# Autodesk Inventor assembly: Пустой корпус
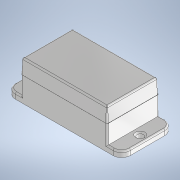
[picture p0: Inventor's stored thumbnail of the model, 180x180]
Saved by Autodesk Inventor 2022 (Build 260153000, 153)
## iProperties
Created: 2022-01-11
Part Number: Пустой корпус
Document SubType Name: Assembly
Designer: m
Author: m
## Documents named in this file (3)
- D:\my_projects\Curse\3D\Сборка\Пустой корпус.iam
- D:\my_projects\Curse\3D\Сборка\case_down.ipt
- D:\my_projects\Curse\3D\Сборка\case_up.ipt
## Components (2 placed, 2 different names)
1. case_down:1 — Совмещение:1, Совмещение:2
2. case_up:1 — Совмещение:1, Совмещение:2
## Relationships (2: Mate 2)
- Совмещение:1 [Mate]: case_down:1 ↔ case_up:1
- Совмещение:2 [Mate]: case_down:1 ↔ case_up:1
